# Autodesk Inventor assembly: Stewart-Base-KST-DS215
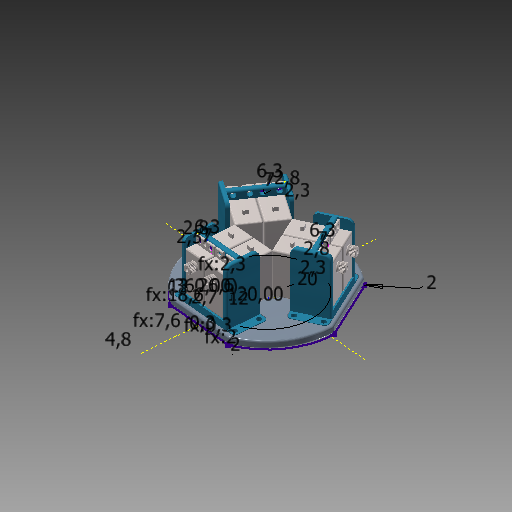
[picture p0: Inventor's stored thumbnail of the model, 512x512]
Saved by Autodesk Inventor 2018.2 (Build 222227000, 227)
## iProperties
Created: 2018-02-24
Part Number: Stewart-Base-KST-DS215
Material: Generisch
Document SubType Name: Assembly
Designer: JochenAlt
Author: JochenAlt
## Documents named in this file (4)
- D:\Projects\Donna\CAD\KST DS215MG\Stewart-Base-KST-DS215.iam
- D:\Projects\Donna\CAD\KST DS215MG\Stewart-Platform-Base-KST-DS215MG.ipt
- D:\Projects\Donna\CAD\KST DS215MG\Stewart-Base-Servo-Holder-KST-DS215.ipt
- D:\Projects\Donna\CAD\KST DS215MG\Servo-KST-DS215MG.ipt
## Components (10 placed, 3 different names)
1. Stewart-Platform-Base-KST-DS215MG:1 — Passend:2, Passend:3, Passend:4, Passend:6, Passend:23, Passend:24, Passend:25, Passend:26, Passend:27
2. Body-Servo-Holder-KST-DS215:1 — Passend:6, Passend:7, Passend:9, Passend:23, Passend:32, Passend:33
3. Servo-KST-DS215MG:1 — Passend:7, Passend:32
4. Servo-KST-DS215MG:2 — Passend:9, Passend:33
5. Body-Servo-Holder-KST-DS215:2 — Passend:17, Passend:18, Passend:24, Passend:25, Passend:30, Passend:31
6. Body-Servo-Holder-KST-DS215:3 — Passend:15, Passend:16, Passend:26, Passend:27, Passend:28, Passend:29
7. Servo-KST-DS215MG:3 — Passend:16, Passend:29
8. Servo-KST-DS215MG:4 — Passend:15, Passend:28
9. Servo-KST-DS215MG:5 — Passend:18, Passend:30
10. Servo-KST-DS215MG:6 — Passend:17, Passend:31
## Relationships (21: Mate 21)
- Passend:2 [Mate]: Stewart-Platform-Base-KST-DS215MG:1
- Passend:3 [Mate]: Stewart-Platform-Base-KST-DS215MG:1
- Passend:4 [Mate]: Stewart-Platform-Base-KST-DS215MG:1
- Passend:6 [Mate]: Stewart-Platform-Base-KST-DS215MG:1 ↔ Body-Servo-Holder-KST-DS215:1
- Passend:7 [Mate]: Body-Servo-Holder-KST-DS215:1 ↔ Servo-KST-DS215MG:1
- Passend:9 [Mate]: Body-Servo-Holder-KST-DS215:1 ↔ Servo-KST-DS215MG:2
- Passend:15 [Mate]: Body-Servo-Holder-KST-DS215:3 ↔ Servo-KST-DS215MG:4
- Passend:16 [Mate]: Body-Servo-Holder-KST-DS215:3 ↔ Servo-KST-DS215MG:3
- Passend:17 [Mate]: Body-Servo-Holder-KST-DS215:2 ↔ Servo-KST-DS215MG:6
- Passend:18 [Mate]: Body-Servo-Holder-KST-DS215:2 ↔ Servo-KST-DS215MG:5
- Passend:23 [Mate]: Stewart-Platform-Base-KST-DS215MG:1 ↔ Body-Servo-Holder-KST-DS215:1
- Passend:24 [Mate]: Stewart-Platform-Base-KST-DS215MG:1 ↔ Body-Servo-Holder-KST-DS215:2
- Passend:25 [Mate]: Stewart-Platform-Base-KST-DS215MG:1 ↔ Body-Servo-Holder-KST-DS215:2
- Passend:26 [Mate]: Stewart-Platform-Base-KST-DS215MG:1 ↔ Body-Servo-Holder-KST-DS215:3
- Passend:27 [Mate]: Stewart-Platform-Base-KST-DS215MG:1 ↔ Body-Servo-Holder-KST-DS215:3
- Passend:28 [Mate]: Body-Servo-Holder-KST-DS215:3 ↔ Servo-KST-DS215MG:4
- Passend:29 [Mate]: Body-Servo-Holder-KST-DS215:3 ↔ Servo-KST-DS215MG:3
- Passend:30 [Mate]: Body-Servo-Holder-KST-DS215:2 ↔ Servo-KST-DS215MG:5
- Passend:31 [Mate]: Body-Servo-Holder-KST-DS215:2 ↔ Servo-KST-DS215MG:6
- Passend:32 [Mate]: Body-Servo-Holder-KST-DS215:1 ↔ Servo-KST-DS215MG:1
- Passend:33 [Mate]: Body-Servo-Holder-KST-DS215:1 ↔ Servo-KST-DS215MG:2
